# Autodesk Inventor assembly: Assembly1
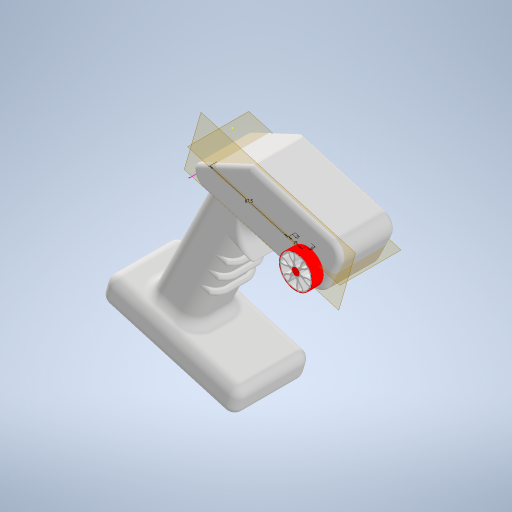
[picture p0: Inventor's stored thumbnail of the model, 512x512]
Saved by Autodesk Inventor 2023 (Build 270158000, 158)
## iProperties
Created: 2023-01-31
Part Number: Assembly1
Document SubType Name: Assembly
Designer: oktay
Author: oktay
## Documents named in this file (6)
- C:\Users\ycsyy\Desktop\HARİKA KUMANDA TASARIMI\Assembly1.iam
- C:\Users\ycsyy\Desktop\HARİKA KUMANDA TASARIMI\Part4.ipt
- C:\Users\ycsyy\Desktop\HARİKA KUMANDA TASARIMI\Part6.ipt
- C:\Users\ycsyy\Desktop\HARİKA KUMANDA TASARIMI\kumandaiç.ipt
- C:\Users\ycsyy\Desktop\HARİKA KUMANDA TASARIMI\kumandadış.ipt
- C:\Users\ycsyy\Desktop\HARİKA KUMANDA TASARIMI\tetik2.ipt
## Components (5 placed, 5 different names)
1. Part4:1 — Mate:1
2. Part6:1 — Mate:1, Mate:6, Mate:7, Rotational:1
3. kumandaiç:1 — Mate:4, Mate:5
4. kumandadış:2 — Mate:4, Mate:5, Mate:6, Mate:7
5. tetik2:1 — Rotational:1
## Relationships (6: Mate 5, RevoluteJoint 1)
- Mate:1: Part4:1 ↔ Part6:1
- Mate:4: kumandaiç:1 ↔ kumandadış:2
- Mate:5: kumandaiç:1 ↔ kumandadış:2
- Mate:6: Part6:1 ↔ kumandadış:2
- Mate:7: Part6:1 ↔ kumandadış:2
- Rotational:1 [RevoluteJoint]: Part6:1 ↔ tetik2:1
